# Autodesk Inventor assembly: Reprinter
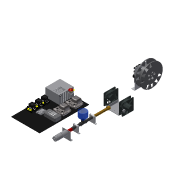
[picture p0: Inventor's stored thumbnail of the model, 180x180]
Saved by Autodesk Inventor 2014 SP1 (Build 180222100, 222)
## iProperties
Created: 2014-11-19
Part Number: Reprinter
Document SubType Name: Assembly
Designer: AlecShufelt
Mass: 4078.47 g
Surface Area: 15412.2 cm^2
Volume: 3707.34 cm^3
Density: 1.10011 g/cm^3
Author: AlecShufelt
## Documents named in this file (16)
- C:\Users\AlecShufelt\Documents\Drafting\CEMS Research\Prototype 2.0\Reprinter.iam
- C:\Users\AlecShufelt\Documents\Drafting\CEMS Research\Prototype 2.0\Puller Mechnaism.iam
- C:\Users\AlecShufelt\Documents\Drafting\CEMS Research\Prototype 2.0\Power Supply.ipt
- C:\Users\AlecShufelt\Documents\Drafting\CEMS Research\Prototype 2.0\Button.ipt
- C:\Users\AlecShufelt\Documents\Drafting\CEMS Research\Prototype 2.0\Spooling Mech.iam
- C:\Users\AlecShufelt\Documents\Drafting\CEMS Research\Prototype 2.0\Board.ipt
- C:\Users\AlecShufelt\Documents\Drafting\CEMS Research\Prototype 2.0\Victor884.iam
- C:\Users\AlecShufelt\Documents\Drafting\CEMS Research\Prototype 2.0\Cooling Mechanism.iam
- C:\Users\AlecShufelt\Documents\Drafting\CEMS Research\Prototype 2.0\Jaguar main enclosure.ipt
- C:\Users\AlecShufelt\Documents\Drafting\CEMS Research\Prototype 2.0\Wheel.ipt
- C:\Users\AlecShufelt\Documents\Drafting\CEMS Research\Prototype 2.0\Keypad.ipt
- C:\Users\AlecShufelt\Documents\Drafting\CEMS Research\Prototype 2.0\Extruder Mechanism.iam
- C:\Users\AlecShufelt\Documents\Drafting\CEMS Research\Prototype 2.0\Imported Components\arduino uno\arduino uno.iam
- C:\Users\AlecShufelt\Documents\Drafting\CEMS Research\Prototype 2.0\Part155.ipt
- C:\Users\AlecShufelt\Documents\Drafting\CEMS Research\Prototype 2.0\Imported Components\PG-71-am-0914\PG-71-am-0914.ipt
- C:\Users\AlecShufelt\Documents\Drafting\CEMS Research\Prototype 2.0\Part157.ipt
## Components (18 placed, 15 different names)
1. Puller Mechnaism:1 [sub-assembly] — Flush:11
2. Power Supply:1 — Flush:1, Flush:2, Mate:1, Flush:4
3. Button:1 — Flush:1, Flush:2
4. Spooling Mech:1 [sub-assembly] — Insert:1, Flush:13
5. Board:1 — Mate:1, Flush:4, Mate:2, Mate:3, Mate:4, Mate:5, Mate:6, Mate:8
6. Victor884:1 [sub-assembly] — Mate:2, Flush:5, Flush:6
7. Victor884:2 [sub-assembly] — Mate:3, Flush:6
8. Victor884:3 [sub-assembly] — Mate:4, Flush:5
9. Cooling Mechanism:1 [sub-assembly] — Flush:12, Mate:10
10. Jaguar main enclosure:1 — Mate:5, Flush:7
11. Jaguar main enclosure:2 — Mate:6, Flush:7
12. Wheel:1 — Insert:1
13. Keypad:1 — Mate:8
14. arduino uno:3 [sub-assembly]
15. Extruder Mechanism:1 [sub-assembly] — Flush:11, Insert:2, Flush:12, Flush:13, Mate:10, Flush:14
16. Part155:1 — Insert:2, Insert:3
17. PG-71-am-0914:1 — Insert:3, Insert:4
18. Part157:1 — Insert:4, Flush:14
## Relationships (23: Flush 10, Mate 9, Insert 4)
- Flush:1 (29.6215 mm): Power Supply:1 ↔ Button:1
- Flush:2 (29.7942 mm): Power Supply:1 ↔ Button:1
- Mate:1: Power Supply:1 ↔ Board:1
- Flush:4: Power Supply:1 ↔ Board:1
- Mate:2: Board:1 ↔ Victor884:1
- Mate:3: Board:1 ↔ Victor884:2
- Mate:4: Board:1 ↔ Victor884:3
- Flush:5: Victor884:1 ↔ Victor884:3
- Flush:6: Victor884:1 ↔ Victor884:2
- Mate:5: Board:1 ↔ Jaguar main enclosure:1
- Mate:6: Board:1 ↔ Jaguar main enclosure:2
- Flush:7: Jaguar main enclosure:1 ↔ Jaguar main enclosure:2
- Insert:1 (-38.1 mm): Spooling Mech:1 ↔ Wheel:1
- Mate:8: Board:1 ↔ Keypad:1
- [Mate]: Board:1 ↔ arduino uno:3
- Flush:11: Puller Mechnaism:1 ↔ Extruder Mechanism:1
- Insert:2: Extruder Mechanism:1 ↔ Part155:1
- Insert:3: Part155:1 ↔ PG-71-am-0914:1
- Flush:12: Cooling Mechanism:1 ↔ Extruder Mechanism:1
- Flush:13: Spooling Mech:1 ↔ Extruder Mechanism:1
- Mate:10 (101.6 mm): Cooling Mechanism:1 ↔ Extruder Mechanism:1
- Insert:4: PG-71-am-0914:1 ↔ Part157:1
- Flush:14: Extruder Mechanism:1 ↔ Part157:1
